# Autodesk Inventor assembly: Assembly_TOTEM_XY_Hi2_Module
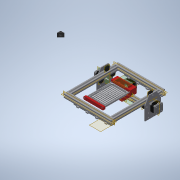
[picture p0: Inventor's stored thumbnail of the model, 180x180]
Saved by Autodesk Inventor 2022 (Build 260153000, 153)
## iProperties
Created: 2021-10-12
Part Number: Assembly_TOTEM_XY_Hi2_Module
Document SubType Name: Assembly
Designer: diederichbenedict
Author: diederichbenedict
## Documents named in this file (7)
- C:\Users\diederichbenedict\Dropbox\Dokumente\Promotion\PROJECTS\UC2\02_CAD\INVENTOR\uc2_v3\Assembly_TOTEM_XY_Hi2_Module.iam
- C:\Users\diederichbenedict\Dropbox\Dokumente\Promotion\PROJECTS\UC2\02_CAD\INVENTOR\uc2_v3\Neje_puzzle_adapterplate_v3.ipt
- C:\Users\diederichbenedict\Dropbox\Dokumente\Promotion\PROJECTS\UC2\02_CAD\INVENTOR\uc2_v3\TOTEM_Slider_Y.iam
- C:\Users\diederichbenedict\Dropbox\Dokumente\Promotion\PROJECTS\UC2\02_CAD\INVENTOR\uc2_v3\TOTEM_Slider_X.iam
- C:\Users\diederichbenedict\Dropbox\Dokumente\Promotion\PROJECTS\UC2\02_CAD\INVENTOR\uc2_v3\00_VSlot_20mm_200mm.ipt
- C:\Users\diederichbenedict\Dropbox\Dokumente\Promotion\PROJECTS\UC2\02_CAD\INVENTOR\uc2_v3\00_VSlot_20mm_250mm.ipt
- C:\Users\diederichbenedict\Dropbox\Dokumente\Promotion\PROJECTS\UC2\02_CAD\INVENTOR\uc2_v3\00_VSlot_90degree_bracket.ipt
## Components (11 placed, 6 different names)
1. TOTEM_Slider_X:1 [sub-assembly] — Flush:10, Insert:2, Angle:3
2. TOTEM_Slider_Y:1 [sub-assembly] — Flush:14, Flush:13
3. 00_VSlot_20mm_200mm:1 — Flush:10
4. 00_VSlot_20mm_250mm:2
5. 00_VSlot_20mm_200mm:2 — Flush:11
6. 00_VSlot_20mm_250mm:1
7. Neje_puzzle_adapterplate_v3:2
8. Neje_puzzle_adapterplate_v3:1
9. 00_VSlot_90degree_bracket:1
10. TOTEM_Slider_X:2 [sub-assembly] — Flush:11, Insert:1
11. 00_VSlot_20mm_250mm:3 — Insert:1, Insert:2, Angle:3, Flush:14, Flush:13
## Relationships (23: Flush 12, Mate 7, Angle 2, Insert 2)
- [Flush]: 00_VSlot_20mm_200mm:1 ↔ 00_VSlot_20mm_250mm:1
- [Mate]: 00_VSlot_20mm_200mm:1 ↔ 00_VSlot_20mm_250mm:1
- [Flush]: 00_VSlot_20mm_200mm:1 ↔ 00_VSlot_20mm_250mm:1
- [Mate]: 00_VSlot_20mm_200mm:1 ↔ 00_VSlot_20mm_250mm:2
- [Flush]: 00_VSlot_20mm_200mm:1 ↔ 00_VSlot_20mm_250mm:2
- [Flush]: 00_VSlot_20mm_200mm:1 ↔ 00_VSlot_20mm_250mm:2
- [Flush]: 00_VSlot_20mm_200mm:2 ↔ 00_VSlot_20mm_250mm:1
- [Mate]: 00_VSlot_20mm_200mm:2 ↔ 00_VSlot_20mm_250mm:1
- [Flush]: 00_VSlot_20mm_200mm:2 ↔ 00_VSlot_20mm_250mm:1
- Flush:10: TOTEM_Slider_X:1 ↔ 00_VSlot_20mm_200mm:1
- [Mate] (1 mm): TOTEM_Slider_X:1 ↔ 00_VSlot_20mm_200mm:1
- Flush:11: 00_VSlot_20mm_200mm:2 ↔ TOTEM_Slider_X:2
- [Mate] (1 mm): 00_VSlot_20mm_200mm:2 ↔ TOTEM_Slider_X:2
- [Mate]: 00_VSlot_20mm_200mm:2 ↔ Neje_puzzle_adapterplate_v3:2
- [Angle] (90 deg): 00_VSlot_20mm_200mm:2 ↔ Neje_puzzle_adapterplate_v3:2
- [Flush]: 00_VSlot_20mm_250mm:2 ↔ Neje_puzzle_adapterplate_v3:2
- [Flush]: 00_VSlot_20mm_250mm:1 ↔ Neje_puzzle_adapterplate_v3:1
- [Mate]: 00_VSlot_20mm_250mm:1 ↔ Neje_puzzle_adapterplate_v3:1
- Insert:1 (1 mm): TOTEM_Slider_X:2 ↔ 00_VSlot_20mm_250mm:3
- Insert:2 (1 mm): TOTEM_Slider_X:1 ↔ 00_VSlot_20mm_250mm:3
- Angle:3 (180 deg): TOTEM_Slider_X:1 ↔ 00_VSlot_20mm_250mm:3
- Flush:14: TOTEM_Slider_Y:1 ↔ 00_VSlot_20mm_250mm:3
- Flush:13: TOTEM_Slider_Y:1 ↔ 00_VSlot_20mm_250mm:3
